# Autodesk Inventor assembly: 110-02
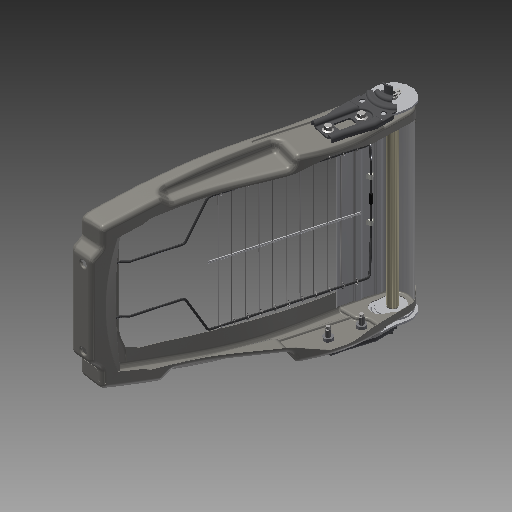
[picture p0: Inventor's stored thumbnail of the model, 512x512]
Saved by Autodesk Inventor 2019 (Build 230136000, 136)
## iProperties
Company: Autodesk Inc.
Created: 2007-12-26
Part Number: 110-02
Document SubType Name: Assembly
Designer: Autodesk Inc.
Mass: 4218.81 g
Surface Area: 7754.19 cm^2
Volume: 539.848 cm^3
Density: 7.81482 g/cm^3
Description: BACK FRAME MAIN ASSEMBLY
Component Category: Back Component
Author: Inventor
## Documents named in this file (19)
- C:\TEMP\Car Seat\Workspace\Back Frame Main Assembly.iam
- C:\TEMP\Car Seat\Workspace\Spring Bracket R.ipt
- C:\TEMP\Car Seat\Workspace\Spring Bracket L.ipt
- C:\TEMP\Car Seat\Workspace\Back Wire R.ipt
- C:\TEMP\Car Seat\Workspace\Back Wire L.ipt
- C:\TEMP\Car Seat\Workspace\Seat Pivot Rod.ipt
- C:\TEMP\Car Seat\Workspace\Pivot Cam Bushing.ipt
- C:\TEMP\Car Seat\Workspace\Back Pivot Plate.ipt
- C:\TEMP\Car Seat\Workspace\Back Member R.ipt
- C:\TEMP\Car Seat\Workspace\Back Member L.ipt
- C:\TEMP\Car Seat\Workspace\Spring Bracket Bolt.ipt
- C:\TEMP\Car Seat\Workspace\Spring Bracket Nut.ipt
- C:\TEMP\Car Seat\Workspace\Lower Pan.ipt
- C:\TEMP\Car Seat\Workspace\Top Plate Mount.ipt
- C:\TEMP\Car Seat\Workspace\Back Top Plate.ipt
- C:\TEMP\Car Seat\Workspace\Wire Clip.ipt
- C:\TEMP\Car Seat\Workspace\Wire Connecting Tube.ipt
- C:\TEMP\Car Seat\Workspace\Wire Connector Bar.ipt
- C:\TEMP\Car Seat\Workspace\Tension Wire.ipt
## Components (37 placed, 18 different names)
1. Top Platform Cross Rod:1 — Mate:1, Flush:1, Flush:2, Insert:1, Insert:2
2. Pivot Cam Bushing:1 — Insert:1, Angle:1, Insert:3
3. Pivot Cam Bushing:2 — Insert:2, Angle:2, Insert:4
4. Back Pivot Plate:1 — Insert:3, Angle:3, Angle:4, Mate:2
5. Back Pivot Plate:2 — Insert:4, Angle:4, Mate:4
6. Spring Bracket R:1 — Mate:2, Mate:3, Angle:5, Angle:6, Insert:5, Mate:6, Insert:7, Insert:8
7. Spring Bracket L:1 — Mate:4, Mate:5, Angle:6, Insert:6, Mate:7, Insert:9, Insert:10
8. Upper Platform R:1 — Insert:5, Mate:6, Insert:11, Insert:12, Angle:7, Mate:13
9. Upper Platform L:1 — Insert:6, Mate:7, Insert:13, Insert:14, Mate:9, Mate:10
10. Spring Bracket Bolt:2 — Insert:8
11. Spring Bracket Bolt:1 — Insert:7
12. Spring Bracket Bolt:3 — Insert:9
13. Spring Bracket Bolt:4 — Insert:10
14. Spring Bracket Nut:1 — Insert:11
15. Spring Bracket Nut:2 — Insert:12
16. Spring Bracket Nut:3 — Insert:13
17. Spring Bracket Nut:4 — Insert:14
18. Upper Platform Base:1 — Flush:3, Mate:8, Angle:7, Mate:16, Mate:17, Mate:18, Mate:19
19. Upper Platform Cap:1 — Flush:4, Mate:9, Mate:10, Mate:12
20. Upper Platform Rear:1 — Mate:11, Mate:12, Mate:13, Mate:21, Mate:22, Mate:24, Mate:25
21. Tension Cage Clip:2 — Mate:16, Mate:18, Angle:8, Mate:20
22. Tension Cage Clip:1 — Mate:17, Mate:19, Angle:9, Mate:23
23. Tension Cage R:1 — Mate:20, Mate:21, Mate:22, Mate:27, Mate:28, Flush:6, Mate:29
24. Tension Cage L:1 — Mate:23, Mate:24, Mate:25
25. Tension Cage Link:1 — Mate:26, Mate:27
26. Wire Connector Bar:1 — Mate:28, Flush:6, Mate:29, Flush:7, Mate:30, Angle:10
27. Tension Wire:1 — Flush:7, Mate:30, Angle:10
28. Tension Wire:2
29. Tension Wire:3
30. Tension Wire:4
31. Tension Wire:5
32. Tension Wire:6
33. Tension Wire:7
34. Tension Wire:8
35. Tension Wire:9
36. Tension Wire:10
37. Tension Wire:11
## Component patterns: (11 elements, first: Tension Wire:1)
## Relationships (58: Mate 28, Insert 14, Angle 10, Flush 6)
- Mate:1: Top Platform Cross Rod:1
- Flush:1: Top Platform Cross Rod:1
- Flush:2: Top Platform Cross Rod:1
- Insert:1: Top Platform Cross Rod:1 ↔ Pivot Cam Bushing:1
- Insert:2: Top Platform Cross Rod:1 ↔ Pivot Cam Bushing:2
- Angle:1 (180 deg): Pivot Cam Bushing:1
- Angle:2 (0 deg): Pivot Cam Bushing:2
- Insert:3 (4.5 mm): Pivot Cam Bushing:1 ↔ Back Pivot Plate:1
- Angle:3 (0 deg): Back Pivot Plate:1
- Insert:4 (4.5 mm): Pivot Cam Bushing:2 ↔ Back Pivot Plate:2
- Angle:4 (180 deg): Back Pivot Plate:1 ↔ Back Pivot Plate:2
- Mate:2: Back Pivot Plate:1 ↔ Spring Bracket R:1
- Mate:3: Spring Bracket R:1
- Angle:5 (180 deg): Spring Bracket R:1
- Mate:4: Back Pivot Plate:2 ↔ Spring Bracket L:1
- Mate:5: Spring Bracket L:1
- Angle:6 (0 deg): Spring Bracket R:1 ↔ Spring Bracket L:1
- Insert:5: Spring Bracket R:1 ↔ Upper Platform R:1
- Mate:6: Spring Bracket R:1 ↔ Upper Platform R:1
- Insert:6: Spring Bracket L:1 ↔ Upper Platform L:1
- Mate:7: Spring Bracket L:1 ↔ Upper Platform L:1
- Insert:7: Spring Bracket R:1 ↔ Spring Bracket Bolt:1
- Insert:8: Spring Bracket R:1 ↔ Spring Bracket Bolt:2
- Insert:9: Spring Bracket L:1 ↔ Spring Bracket Bolt:3
- Insert:10: Spring Bracket L:1 ↔ Spring Bracket Bolt:4
- Insert:11: Upper Platform R:1 ↔ Spring Bracket Nut:1
- Insert:12: Upper Platform R:1 ↔ Spring Bracket Nut:2
- Insert:13: Upper Platform L:1 ↔ Spring Bracket Nut:3
- Insert:14: Upper Platform L:1 ↔ Spring Bracket Nut:4
- Flush:3: Upper Platform Base:1
- Mate:8: Upper Platform Base:1
- Angle:7 (0 deg): Upper Platform R:1 ↔ Upper Platform Base:1
- Flush:4: Upper Platform Cap:1
- Mate:9: Upper Platform L:1 ↔ Upper Platform Cap:1
- Mate:10: Upper Platform L:1 ↔ Upper Platform Cap:1
- Mate:11: Upper Platform Rear:1
- Mate:12: Upper Platform Cap:1 ↔ Upper Platform Rear:1
- Mate:13: Upper Platform R:1 ↔ Upper Platform Rear:1
- Mate:16: Upper Platform Base:1 ↔ Tension Cage Clip:2
- Mate:17: Upper Platform Base:1 ↔ Tension Cage Clip:1
- Mate:18: Upper Platform Base:1 ↔ Tension Cage Clip:2
- Mate:19: Upper Platform Base:1 ↔ Tension Cage Clip:1
- Angle:8 (90 deg): Tension Cage Clip:2
- Angle:9 (90 deg): Tension Cage Clip:1
- Mate:20: Tension Cage Clip:2 ↔ Tension Cage R:1
- Mate:21: Upper Platform Rear:1 ↔ Tension Cage R:1
- Mate:22: Upper Platform Rear:1 ↔ Tension Cage R:1
- Mate:23: Tension Cage Clip:1 ↔ Tension Cage L:1
- Mate:24: Upper Platform Rear:1 ↔ Tension Cage L:1
- Mate:25: Upper Platform Rear:1 ↔ Tension Cage L:1
- Mate:26: Tension Cage Link:1
- Mate:27: Tension Cage R:1 ↔ Tension Cage Link:1
- Mate:28 (-2.825 mm): Tension Cage R:1 ↔ Wire Connector Bar:1
- Flush:6 (195 mm): Tension Cage R:1 ↔ Wire Connector Bar:1
- Mate:29 (129.703 mm): Tension Cage R:1 ↔ Wire Connector Bar:1
- Flush:7: Wire Connector Bar:1 ↔ Tension Wire:1
- Mate:30: Wire Connector Bar:1 ↔ Tension Wire:1
- Angle:10 (0 deg): Wire Connector Bar:1 ↔ Tension Wire:1
